# Autodesk Inventor assembly: AM14U2 Half Long
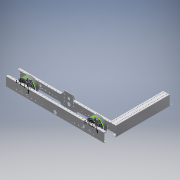
[picture p0: Inventor's stored thumbnail of the model, 180x180]
Saved by Autodesk Inventor 2016 (Build 200138000, 138)
## iProperties
Created: 2014-12-16
Part Number: AM14U2 Half Long
Document SubType Name: Assembly
Designer: Philip
Author: Philip
## Documents named in this file (7)
- C:\Users\Administrator\Desktop\3192CAD\InitialRobotProto\amparts\AM14U2 Half Long.iam
- C:\Users\Administrator\Desktop\3192CAD\InitialRobotProto\amparts\am-2951 AM14U2 Outside Sheet.ipt
- C:\Users\Administrator\Desktop\3192CAD\InitialRobotProto\amparts\am-2952 AM14U2 Inside Sheet.ipt
- C:\Users\Administrator\Desktop\3192CAD\InitialRobotProto\amparts\10-32x0625 with nut.iam
- C:\Users\Administrator\Desktop\3192CAD\InitialRobotProto\amparts\am-2953 AM14U2 End Sheet Square.ipt
- C:\Users\Administrator\Desktop\3192CAD\InitialRobotProto\WheelPart.ipt
- C:\Users\Administrator\Desktop\3192CAD\InitialRobotProto\DBK_C-Channel_Tiny.ipt
## Components (9 placed, 7 different names)
1. am-2951 AM14U2 Outside Sheet_9 — Mate:4, Mate:5, Mate:6, Mate:7, Mate:8, Mate:9, Mate:12, Mate:13
2. am-2952 AM14U2 Inside Sheet_10 — Mate:1, Mate:2, Mate:3, Mate:6, Mate:7, Mate:10, Mate:11
3. 10-32x0625 with nut_32 [sub-assembly]
4. 10-32x0625 with nut_33 [sub-assembly]
5. am-2953 AM14U2 End Sheet Square:1 — Mate:1, Mate:2, Mate:3
6. WheelPart:1 — Mate:4
7. WheelPart:2 — Mate:5
8. DBK_C-Channel_Tiny:1 — Mate:8, Mate:9, Mate:10
9. DBK_C-Channel_Tiny:2 — Mate:11, Mate:12, Mate:13
## Relationships (13: Mate 13)
- Mate:1: am-2952 AM14U2 Inside Sheet_10 ↔ am-2953 AM14U2 End Sheet Square:1
- Mate:2: am-2952 AM14U2 Inside Sheet_10 ↔ am-2953 AM14U2 End Sheet Square:1
- Mate:3: am-2952 AM14U2 Inside Sheet_10 ↔ am-2953 AM14U2 End Sheet Square:1
- Mate:4: am-2951 AM14U2 Outside Sheet_9 ↔ WheelPart:1
- Mate:5: am-2951 AM14U2 Outside Sheet_9 ↔ WheelPart:2
- Mate:6: am-2951 AM14U2 Outside Sheet_9 ↔ am-2952 AM14U2 Inside Sheet_10
- Mate:7: am-2951 AM14U2 Outside Sheet_9 ↔ am-2952 AM14U2 Inside Sheet_10
- Mate:8: am-2951 AM14U2 Outside Sheet_9 ↔ DBK_C-Channel_Tiny:1
- Mate:9: am-2951 AM14U2 Outside Sheet_9 ↔ DBK_C-Channel_Tiny:1
- Mate:10: am-2952 AM14U2 Inside Sheet_10 ↔ DBK_C-Channel_Tiny:1
- Mate:11: am-2952 AM14U2 Inside Sheet_10 ↔ DBK_C-Channel_Tiny:2
- Mate:12: am-2951 AM14U2 Outside Sheet_9 ↔ DBK_C-Channel_Tiny:2
- Mate:13: am-2951 AM14U2 Outside Sheet_9 ↔ DBK_C-Channel_Tiny:2
